# Autodesk Inventor assembly: Alu Ramen
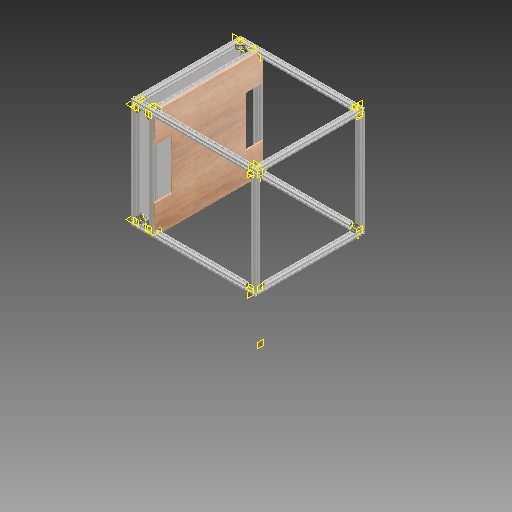
[picture p0: Inventor's stored thumbnail of the model, 512x512]
Saved by Autodesk Inventor 2018 (Build 220112000, 112)
## iProperties
Part Number: Alu Ramen
Material: Generisch
Document SubType Name: Assembly
Designer: Till
Author: Till
## Documents named in this file (6)
- C:\Users\Till\Dropbox\Ultibox\ultibox\cad\Alu Ramen.iam
- C:\Users\Till\Dropbox\Ultibox\ultibox\cad\500mm.ipt
- C:\Users\Till\Dropbox\Ultibox\ultibox\cad\400mm.ipt
- C:\Users\Till\Dropbox\Ultibox\ultibox\cad\corner pieces + screw.iam
- C:\Users\Till\Dropbox\Ultibox\ultibox\cad\ground plate.ipt
- C:\Users\Till\Dropbox\DIY\CoreBot\STL files\middle plate.ipt
## Components (50 placed, 19 different names)
1. ground plate:1 — Passend:80, Passend:81
2. middle plate:1 — Fluchtend:143
3. X bottom front — Passend:27, Fluchtend:25, Fluchtend:26, Passend:63, Passend:64, Passend:65, Fluchtend:107, Fluchtend:108, Fluchtend:113, Fluchtend:116, Fluchtend:117, Fluchtend:118
4. X bottom back — Fluchtend:27, Fluchtend:28, Passend:28, Passend:57, Passend:59, Fluchtend:101, Fluchtend:102, Fluchtend:105, Fluchtend:106, Passend:81
5. Y bottom right — Passend:10, Fluchtend:15, Fluchtend:16, Passend:43, Passend:61, Passend:66, Passend:67, Fluchtend:99, Fluchtend:100, Fluchtend:109, Fluchtend:110, Fluchtend:111, Fluchtend:112, Passend:80
6. Y bottom left — Passend:29, Fluchtend:29, Fluchtend:30, Passend:56, Passend:62, Fluchtend:103, Fluchtend:104, Fluchtend:114, Fluchtend:115
7. X middle front — Passend:44, Fluchtend:74, Fluchtend:75, Fluchtend:77, Passend:53, Passend:54, Fluchtend:82, Fluchtend:83, Fluchtend:84
8. X middle back — Passend:46, Fluchtend:78, Fluchtend:79, Passend:49, Passend:50, Fluchtend:89, Fluchtend:90, Fluchtend:93, Fluchtend:94, Passend:58, Passend:60, Fluchtend:95, Fluchtend:96, Fluchtend:97, Fluchtend:98
9. Y middle right — Passend:42, Fluchtend:73, Passend:43, Fluchtend:75, Passend:47, Fluchtend:80, Fluchtend:81, Passend:48, Fluchtend:91, Fluchtend:92, Fluchtend:143
10. Y middle left — Passend:45, Fluchtend:76, Fluchtend:77, Fluchtend:79, Passend:51, Passend:52, Fluchtend:85, Fluchtend:86, Fluchtend:87, Fluchtend:88
11. X top front — Passend:5, Fluchtend:5, Fluchtend:6, Passend:8, Fluchtend:11, Fluchtend:12, Passend:73, Passend:74, Passend:76, Fluchtend:119, Fluchtend:120, Fluchtend:121, Fluchtend:122, Fluchtend:129, Fluchtend:130
12. X top back — Passend:6, Fluchtend:7, Fluchtend:8, Passend:7, Fluchtend:9, Fluchtend:10, Passend:68, Passend:69, Passend:78, Passend:79, Fluchtend:131, Fluchtend:132, Fluchtend:133, Fluchtend:134, Fluchtend:137, Fluchtend:138, Fluchtend:141, Fluchtend:142
13. Y top right — Passend:1, Fluchtend:1, Fluchtend:2, Passend:4, Fluchtend:3, Fluchtend:4, Passend:70, Passend:71, Passend:72, Fluchtend:125, Fluchtend:126, Fluchtend:127, Fluchtend:128, Fluchtend:135, Fluchtend:136
14. Y top left — Passend:9, Fluchtend:13, Fluchtend:14, Passend:75, Passend:77, Fluchtend:123, Fluchtend:124, Fluchtend:139, Fluchtend:140
15. Z front right — Passend:1, Fluchtend:1, Fluchtend:2, Passend:6, Fluchtend:7, Fluchtend:8, Passend:10, Fluchtend:15, Fluchtend:16, Fluchtend:27, Fluchtend:28, Passend:28, Passend:42, Fluchtend:73
16. Z front left — Passend:7, Fluchtend:9, Fluchtend:10, Passend:29, Fluchtend:29, Fluchtend:30, Passend:46, Fluchtend:78
17. Z back right — Passend:4, Fluchtend:3, Fluchtend:4, Passend:5, Fluchtend:5, Fluchtend:6, Passend:27, Fluchtend:25, Fluchtend:26, Passend:44, Fluchtend:74, Passend:55
18. Z back left — Passend:8, Fluchtend:11, Fluchtend:12, Passend:9, Fluchtend:13, Fluchtend:14, Passend:45, Fluchtend:76
19. corner pieces + screw:21 [sub-assembly] — Passend:78, Fluchtend:137, Fluchtend:138
20. corner pieces + screw:22 [sub-assembly] — Passend:77, Fluchtend:139, Fluchtend:140
21. corner pieces + screw:23 [sub-assembly] — Passend:76, Fluchtend:119, Fluchtend:120
22. corner pieces + screw:24 [sub-assembly] — Passend:79, Fluchtend:141, Fluchtend:142
23. corner pieces + screw:25 [sub-assembly] — Passend:75, Fluchtend:123, Fluchtend:124
24. corner pieces + screw:26 [sub-assembly] — Passend:74, Fluchtend:121, Fluchtend:122
25. corner pieces + screw:27 [sub-assembly] — Passend:72, Fluchtend:127, Fluchtend:128
26. corner pieces + screw:28 [sub-assembly] — Passend:73, Fluchtend:129, Fluchtend:130
27. corner pieces + screw:29 [sub-assembly] — Passend:71, Fluchtend:125, Fluchtend:126
28. corner pieces + screw:30 [sub-assembly] — Passend:70, Fluchtend:135, Fluchtend:136
29. corner pieces + screw:31 [sub-assembly] — Passend:69, Fluchtend:133, Fluchtend:134
30. corner pieces + screw:32 [sub-assembly] — Passend:68, Fluchtend:131, Fluchtend:132
31. corner pieces + screw:1 [sub-assembly] — Passend:51, Fluchtend:87, Fluchtend:88
32. corner pieces + screw:2 [sub-assembly] — Passend:53, Fluchtend:83, Fluchtend:84
33. corner pieces + screw:3 [sub-assembly] — Passend:47, Fluchtend:80, Fluchtend:81
34. corner pieces + screw:4 [sub-assembly] — Passend:52, Fluchtend:85, Fluchtend:86
35. corner pieces + screw:5 [sub-assembly] — Passend:54, Passend:55, Fluchtend:82
36. corner pieces + screw:6 [sub-assembly] — Passend:50, Fluchtend:89, Fluchtend:90
37. corner pieces + screw:7 [sub-assembly] — Passend:49, Fluchtend:93, Fluchtend:94
38. corner pieces + screw:8 [sub-assembly] — Passend:48, Fluchtend:91, Fluchtend:92
39. corner pieces + screw:13 [sub-assembly] — Passend:60, Fluchtend:95, Fluchtend:96
40. corner pieces + screw:14 [sub-assembly] — Passend:58, Fluchtend:97, Fluchtend:98
41. corner pieces + screw:9 [sub-assembly] — Passend:57, Fluchtend:105, Fluchtend:106
42. corner pieces + screw:10 [sub-assembly] — Passend:56, Fluchtend:103, Fluchtend:104
43. corner pieces + screw:11 [sub-assembly] — Passend:59, Fluchtend:101, Fluchtend:102
44. corner pieces + screw:12 [sub-assembly] — Passend:61, Fluchtend:99, Fluchtend:100
45. corner pieces + screw:15 [sub-assembly] — Passend:62, Fluchtend:114, Fluchtend:115
46. corner pieces + screw:16 [sub-assembly] — Passend:63, Fluchtend:113, Fluchtend:118
47. corner pieces + screw:17 [sub-assembly] — Passend:64, Fluchtend:116, Fluchtend:117
48. corner pieces + screw:18 [sub-assembly] — Passend:67, Fluchtend:111, Fluchtend:112
49. corner pieces + screw:19 [sub-assembly] — Passend:66, Fluchtend:109, Fluchtend:110
50. corner pieces + screw:20 [sub-assembly] — Passend:65, Fluchtend:107, Fluchtend:108
## Relationships (144: Flush 93, Mate 51)
- Passend:1 [Mate]: Y top right ↔ Z front right
- Fluchtend:1 [Flush]: Y top right ↔ Z front right
- Fluchtend:2 [Flush]: Y top right ↔ Z front right
- Passend:4 [Mate]: Y top right ↔ Z back right
- Fluchtend:3 [Flush]: Y top right ↔ Z back right
- Fluchtend:4 [Flush]: Y top right ↔ Z back right
- Passend:5 [Mate]: X top front ↔ Z back right
- Fluchtend:5 [Flush]: X top front ↔ Z back right
- Fluchtend:6 [Flush]: X top front ↔ Z back right
- Passend:6 [Mate]: X top back ↔ Z front right
- Fluchtend:7 [Flush]: X top back ↔ Z front right
- Fluchtend:8 [Flush]: X top back ↔ Z front right
- Passend:7 [Mate]: X top back ↔ Z front left
- Fluchtend:9 [Flush]: X top back ↔ Z front left
- Fluchtend:10 [Flush]: X top back ↔ Z front left
- Passend:8 [Mate]: X top front ↔ Z back left
- Fluchtend:11 [Flush]: X top front ↔ Z back left
- Fluchtend:12 [Flush]: X top front ↔ Z back left
- Passend:9 [Mate]: Y top left ↔ Z back left
- Fluchtend:13 [Flush]: Y top left ↔ Z back left
- Fluchtend:14 [Flush]: Y top left ↔ Z back left
- Passend:10 [Mate]: Y bottom right ↔ Z front right
- Fluchtend:15 [Flush]: Y bottom right ↔ Z front right
- Fluchtend:16 [Flush]: Y bottom right ↔ Z front right
- Passend:27 [Mate]: X bottom front ↔ Z back right
- Fluchtend:25 [Flush]: X bottom front ↔ Z back right
- Fluchtend:26 [Flush]: X bottom front ↔ Z back right
- Fluchtend:27 [Flush]: X bottom back ↔ Z front right
- Fluchtend:28 [Flush]: X bottom back ↔ Z front right
- Passend:28 [Mate]: X bottom back ↔ Z front right
- Passend:29 [Mate]: Y bottom left ↔ Z front left
- Fluchtend:29 [Flush]: Y bottom left ↔ Z front left
- Fluchtend:30 [Flush]: Y bottom left ↔ Z front left
- Passend:42 [Mate]: Y middle right ↔ Z front right
- Fluchtend:73 [Flush]: Y middle right ↔ Z front right
- Passend:43 [Mate] (50 mm): Y bottom right ↔ Y middle right
- Passend:44 [Mate]: X middle front ↔ Z back right
- Fluchtend:74 [Flush]: X middle front ↔ Z back right
- Fluchtend:75 [Flush]: X middle front ↔ Y middle right
- Passend:45 [Mate]: Y middle left ↔ Z back left
- Fluchtend:76 [Flush]: Y middle left ↔ Z back left
- Fluchtend:77 [Flush]: X middle front ↔ Y middle left
- Passend:46 [Mate]: X middle back ↔ Z front left
- Fluchtend:78 [Flush]: X middle back ↔ Z front left
- Fluchtend:79 [Flush]: X middle back ↔ Y middle left
- Passend:47 [Mate]: Y middle right ↔ corner pieces + screw:3
- Fluchtend:80 [Flush] (1.5 mm): Y middle right ↔ corner pieces + screw:3
- Fluchtend:81 [Flush]: Y middle right ↔ corner pieces + screw:3
- Passend:48 [Mate]: Y middle right ↔ corner pieces + screw:8
- Passend:49 [Mate]: X middle back ↔ corner pieces + screw:7
- Passend:50 [Mate]: X middle back ↔ corner pieces + screw:6
- Passend:51 [Mate]: Y middle left ↔ corner pieces + screw:1
- Passend:52 [Mate]: Y middle left ↔ corner pieces + screw:4
- Passend:53 [Mate]: X middle front ↔ corner pieces + screw:2
- Passend:54 [Mate]: X middle front ↔ corner pieces + screw:5
- Passend:55 [Mate]: Z back right ↔ corner pieces + screw:5
- Fluchtend:82 [Flush] (1.5 mm): X middle front ↔ corner pieces + screw:5
- Fluchtend:83 [Flush]: X middle front ↔ corner pieces + screw:2
- Fluchtend:84 [Flush] (1.5 mm): X middle front ↔ corner pieces + screw:2
- Fluchtend:85 [Flush]: Y middle left ↔ corner pieces + screw:4
- Fluchtend:86 [Flush] (1.5 mm): Y middle left ↔ corner pieces + screw:4
- Fluchtend:87 [Flush]: Y middle left ↔ corner pieces + screw:1
- Fluchtend:88 [Flush] (1.5 mm): Y middle left ↔ corner pieces + screw:1
- Fluchtend:89 [Flush]: X middle back ↔ corner pieces + screw:6
- Fluchtend:90 [Flush] (1.5 mm): X middle back ↔ corner pieces + screw:6
- Fluchtend:91 [Flush]: Y middle right ↔ corner pieces + screw:8
- Fluchtend:92 [Flush] (1.5 mm): Y middle right ↔ corner pieces + screw:8
- Fluchtend:93 [Flush]: X middle back ↔ corner pieces + screw:7
- Fluchtend:94 [Flush] (1.5 mm): X middle back ↔ corner pieces + screw:7
- Passend:56 [Mate]: Y bottom left ↔ corner pieces + screw:10
- Passend:57 [Mate]: X bottom back ↔ corner pieces + screw:9
- Passend:58 [Mate]: X middle back ↔ corner pieces + screw:14
- Passend:59 [Mate]: X bottom back ↔ corner pieces + screw:11
- Passend:60 [Mate]: X middle back ↔ corner pieces + screw:13
- Passend:61 [Mate]: Y bottom right ↔ corner pieces + screw:12
- Passend:62 [Mate]: Y bottom left ↔ corner pieces + screw:15
- Passend:63 [Mate]: X bottom front ↔ corner pieces + screw:16
- Passend:64 [Mate]: X bottom front ↔ corner pieces + screw:17
- Passend:65 [Mate]: X bottom front ↔ corner pieces + screw:20
- Passend:66 [Mate]: Y bottom right ↔ corner pieces + screw:19
- Passend:67 [Mate]: Y bottom right ↔ corner pieces + screw:18
- Fluchtend:95 [Flush]: X middle back ↔ corner pieces + screw:13
- Fluchtend:96 [Flush] (1.5 mm): X middle back ↔ corner pieces + screw:13
- Fluchtend:97 [Flush] (1.5 mm): X middle back ↔ corner pieces + screw:14
- Fluchtend:98 [Flush]: X middle back ↔ corner pieces + screw:14
- Fluchtend:99 [Flush]: Y bottom right ↔ corner pieces + screw:12
- Fluchtend:100 [Flush] (1.5 mm): Y bottom right ↔ corner pieces + screw:12
- Fluchtend:101 [Flush]: X bottom back ↔ corner pieces + screw:11
- Fluchtend:102 [Flush] (1.5 mm): X bottom back ↔ corner pieces + screw:11
- Fluchtend:103 [Flush]: Y bottom left ↔ corner pieces + screw:10
- Fluchtend:104 [Flush] (1.5 mm): Y bottom left ↔ corner pieces + screw:10
- Fluchtend:105 [Flush] (1.5 mm): X bottom back ↔ corner pieces + screw:9
- Fluchtend:106 [Flush]: X bottom back ↔ corner pieces + screw:9
- Fluchtend:107 [Flush]: X bottom front ↔ corner pieces + screw:20
- Fluchtend:108 [Flush] (1.5 mm): X bottom front ↔ corner pieces + screw:20
- Fluchtend:109 [Flush] (1.5 mm): Y bottom right ↔ corner pieces + screw:19
- Fluchtend:110 [Flush]: Y bottom right ↔ corner pieces + screw:19
- Fluchtend:111 [Flush]: Y bottom right ↔ corner pieces + screw:18
- Fluchtend:112 [Flush] (1.5 mm): Y bottom right ↔ corner pieces + screw:18
- Fluchtend:113 [Flush] (1.5 mm): X bottom front ↔ corner pieces + screw:16
- Fluchtend:114 [Flush] (1.5 mm): Y bottom left ↔ corner pieces + screw:15
- Fluchtend:115 [Flush]: Y bottom left ↔ corner pieces + screw:15
- Fluchtend:116 [Flush]: X bottom front ↔ corner pieces + screw:17
- Fluchtend:117 [Flush] (1.5 mm): X bottom front ↔ corner pieces + screw:17
- Fluchtend:118 [Flush]: X bottom front ↔ corner pieces + screw:16
- Passend:68 [Mate]: X top back ↔ corner pieces + screw:32
- Passend:69 [Mate]: X top back ↔ corner pieces + screw:31
- Passend:70 [Mate]: Y top right ↔ corner pieces + screw:30
- Passend:71 [Mate]: Y top right ↔ corner pieces + screw:29
- Passend:72 [Mate]: Y top right ↔ corner pieces + screw:27
- Passend:73 [Mate]: X top front ↔ corner pieces + screw:28
- Passend:74 [Mate]: X top front ↔ corner pieces + screw:26
- Passend:75 [Mate]: Y top left ↔ corner pieces + screw:25
- Passend:76 [Mate]: X top front ↔ corner pieces + screw:23
- Passend:77 [Mate]: Y top left ↔ corner pieces + screw:22
- Passend:78 [Mate]: X top back ↔ corner pieces + screw:21
- Passend:79 [Mate]: X top back ↔ corner pieces + screw:24
- Fluchtend:119 [Flush]: X top front ↔ corner pieces + screw:23
- Fluchtend:120 [Flush] (1.5 mm): X top front ↔ corner pieces + screw:23
- Fluchtend:121 [Flush]: X top front ↔ corner pieces + screw:26
- Fluchtend:122 [Flush] (1.5 mm): X top front ↔ corner pieces + screw:26
- Fluchtend:123 [Flush]: Y top left ↔ corner pieces + screw:25
- Fluchtend:124 [Flush] (1.5 mm): Y top left ↔ corner pieces + screw:25
- Fluchtend:125 [Flush]: Y top right ↔ corner pieces + screw:29
- Fluchtend:126 [Flush] (1.5 mm): Y top right ↔ corner pieces + screw:29
- Fluchtend:127 [Flush]: Y top right ↔ corner pieces + screw:27
- Fluchtend:128 [Flush] (1.5 mm): Y top right ↔ corner pieces + screw:27
- Fluchtend:129 [Flush]: X top front ↔ corner pieces + screw:28
- Fluchtend:130 [Flush] (1.5 mm): X top front ↔ corner pieces + screw:28
- Fluchtend:131 [Flush]: X top back ↔ corner pieces + screw:32
- Fluchtend:132 [Flush] (1.5 mm): X top back ↔ corner pieces + screw:32
- Fluchtend:133 [Flush]: X top back ↔ corner pieces + screw:31
- Fluchtend:134 [Flush] (1.5 mm): X top back ↔ corner pieces + screw:31
- Fluchtend:135 [Flush]: Y top right ↔ corner pieces + screw:30
- Fluchtend:136 [Flush] (1.5 mm): Y top right ↔ corner pieces + screw:30
- Fluchtend:137 [Flush]: X top back ↔ corner pieces + screw:21
- Fluchtend:138 [Flush] (1.5 mm): X top back ↔ corner pieces + screw:21
- Fluchtend:139 [Flush]: Y top left ↔ corner pieces + screw:22
- Fluchtend:140 [Flush] (1.5 mm): Y top left ↔ corner pieces + screw:22
- Fluchtend:141 [Flush]: X top back ↔ corner pieces + screw:24
- Fluchtend:142 [Flush] (1.5 mm): X top back ↔ corner pieces + screw:24
- Passend:80 [Mate] (-4 mm): ground plate:1 ↔ Y bottom right
- Passend:81 [Mate] (-4 mm): ground plate:1 ↔ X bottom back
- Fluchtend:143 [Flush]: middle plate:1 ↔ Y middle right
